# Autodesk Inventor assembly: LINK5
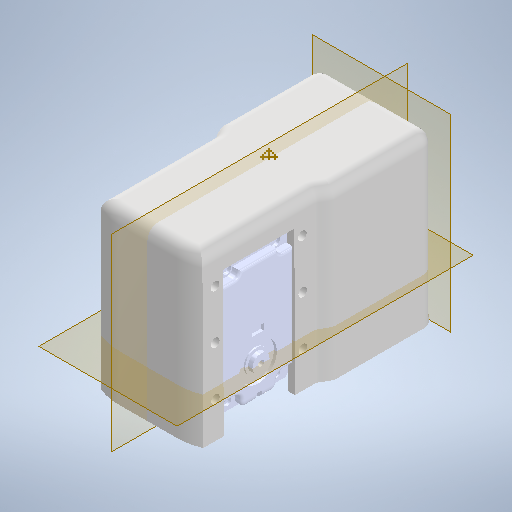
[picture p0: Inventor's stored thumbnail of the model, 512x512]
Saved by Autodesk Inventor 2026.1 (Build 301233020, 233B)
## iProperties
Created: 2025-10-15
Part Number: LINK5
Document SubType Name: Assembly
Designer: wlgns
Author: wlgns
## Documents named in this file (3)
- C:\Users\wlgns\Desktop\project\ARA Project\ARA_CAD_model\ARA_v2\LINK5.iam
- C:\Users\wlgns\Desktop\project\ARA Project\ARA_CAD_model\ARA_v2\ARM_3 SKETCH1.ipt
- C:\Users\wlgns\Desktop\project\ARA Project\ARA_CAD_model\ARA_v2\MX-28T_MIR.ipt
## Components (3 placed, 2 different names)
1. ARM_3 SKETCH1:1 — 메이트:1, 메이트:2, 메이트:3, 메이트:4, 메이트:5, 메이트:6, 메이트:10
2. MX-28T_MIR:1 — 메이트:1, 메이트:2, 메이트:3, 플러쉬:1, 메이트:8, 메이트:9
3. MX-28T_MIR:2 — 메이트:4, 메이트:5, 메이트:6
## Relationships (11: Mate 10, Flush 1)
- 메이트:1 [Mate]: ARM_3 SKETCH1:1 ↔ MX-28T_MIR:1
- 메이트:2 [Mate]: ARM_3 SKETCH1:1 ↔ MX-28T_MIR:1
- 메이트:3 [Mate]: ARM_3 SKETCH1:1 ↔ MX-28T_MIR:1
- 메이트:4 [Mate]: ARM_3 SKETCH1:1 ↔ MX-28T_MIR:2
- 메이트:5 [Mate]: ARM_3 SKETCH1:1 ↔ MX-28T_MIR:2
- 메이트:6 [Mate]: ARM_3 SKETCH1:1 ↔ MX-28T_MIR:2
- 플러쉬:1 [Flush] (1.9 mm): MX-28T_MIR:1
- 메이트:7 [Mate]
- 메이트:8 [Mate]: MX-28T_MIR:1
- 메이트:9 [Mate]: MX-28T_MIR:1
- 메이트:10 [Mate]: ARM_3 SKETCH1:1
